# Autodesk Inventor assembly: AXp4s
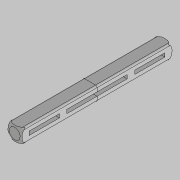
[picture p0: Inventor's stored thumbnail of the model, 180x180]
Saved by Autodesk Inventor 2020 (Build 240168000, 168)
## iProperties
Created: 2019-05-09
Part Number: AXp4s
Document SubType Name: Assembly
Designer: Varga Daniel
Author: Varga Daniel
## Documents named in this file (3)
- C:\!_Dani\!_cloud\OneDrive\!_munka\Revolution\StructuralParts\Axles\AXpXs\AXp4s.iam
- C:\!_Dani\!_cloud\OneDrive\!_munka\Revolution\StructuralParts\Axles\One_sided_axle_base.ipt
- C:\!_Dani\!_cloud\OneDrive\!_munka\Revolution\StructuralParts\Axles\One_sided_axle_base\One_sided_axle_base-20.ipt
## Components (2 placed, 1 different names)
1. One_sided_axle_base-20:1 — Mate:1, Mate:2, Flush:1, Mate:3, Flush:2, Flush:3
2. One_sided_axle_base-20:2 — Mate:3, Flush:2, Flush:3
## Relationships (6: Mate 3, Flush 3)
- Mate:1: One_sided_axle_base-20:1
- Mate:2: One_sided_axle_base-20:1
- Flush:1: One_sided_axle_base-20:1
- Mate:3: One_sided_axle_base-20:1 ↔ One_sided_axle_base-20:2
- Flush:2: One_sided_axle_base-20:1 ↔ One_sided_axle_base-20:2
- Flush:3: One_sided_axle_base-20:1 ↔ One_sided_axle_base-20:2
